# Autodesk Inventor assembly: SoporteBobina_1
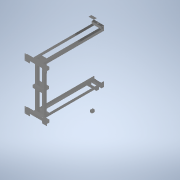
[picture p0: Inventor's stored thumbnail of the model, 180x180]
Saved by Autodesk Inventor 2022 (Build 260153000, 153)
## iProperties
Created: 2022-03-28
Part Number: SoporteBobina_1
Document SubType Name: Assembly
Designer: aarco
Author: aarco
## Documents named in this file (10)
- C:\Users\dovalle\OneDrive - ALTER TECHNOLOGY TÜV NORD, S.A.U\Escritorio\IDOM\REV_3\SoporteBobina_1.iam
- C:\Users\dovalle\OneDrive - ALTER TECHNOLOGY TÜV NORD, S.A.U\Escritorio\IDOM\REV_3\A_1012_40_4.ipt
- C:\Users\dovalle\OneDrive - ALTER TECHNOLOGY TÜV NORD, S.A.U\Escritorio\IDOM\REV_3\C_370_40_2.ipt
- C:\Users\dovalle\OneDrive - ALTER TECHNOLOGY TÜV NORD, S.A.U\Escritorio\IDOM\REV_3\C_156_40_2.ipt
- C:\Users\dovalle\OneDrive - ALTER TECHNOLOGY TÜV NORD, S.A.U\Escritorio\IDOM\REV_3\C_805_40_2.ipt
- C:\Users\dovalle\OneDrive - ALTER TECHNOLOGY TÜV NORD, S.A.U\Escritorio\IDOM\REV_3\Placa_Rueda_105x85_80x60_3.ipt
- C:\Users\dovalle\OneDrive - ALTER TECHNOLOGY TÜV NORD, S.A.U\Escritorio\IDOM\REV_3\C_156_40_20_2.ipt
- C:\Users\dovalle\OneDrive - ALTER TECHNOLOGY TÜV NORD, S.A.U\Escritorio\IDOM\REV_3\C_164_40_4.ipt
- C:\Users\dovalle\OneDrive - ALTER TECHNOLOGY TÜV NORD, S.A.U\Escritorio\IDOM\REV_3\C_45_35_2.ipt
- C:\Users\dovalle\OneDrive - ALTER TECHNOLOGY TÜV NORD, S.A.U\Escritorio\IDOM\REV_3\PlacaSTC-HH20.ipt
## Components (24 placed, 9 different names)
1. A_1012_40_4:1 — Rígido:25, Rígido:29, Coincidencia:6
2. C_370_40_2:1 — Rígido:16, Rígido:19, Rígido:20
3. A_1012_40_4:2 — Rígido:27, Coincidencia:2, Nivelación:2
4. C_370_40_2:2 — Rígido:17, Rígido:18, Rígido:21
5. C_156_40_2:1 — Rígido:1, Rígido:2
6. C_156_40_2:4 — Rígido:5
7. C_156_40_2:5 — Rígido:6
8. C_156_40_2:6 — Rígido:7
9. C_805_40_2:1 — Rígido:2, Rígido:6, Rígido:7
10. C_805_40_2:2 — Rígido:1, Rígido:5, Rígido:22, Rígido:23
11. A_1012_40_4:3 — Rígido:26, Rígido:28, Coincidencia:3, Nivelación:3
12. A_1012_40_4:4 — Rígido:24
13. Placa_Rueda_105x85_80x60_3:1 — Rígido:16
14. Placa_Rueda_105x85_80x60_3:2 — Rígido:17
15. Placa_Rueda_105x85_80x60_3:3 — Rígido:18
16. Placa_Rueda_105x85_80x60_3:4 — Rígido:19
17. C_156_40_20_2:1 — Rígido:20, Rígido:22, Rígido:24, Rígido:25
18. C_156_40_20_2:2 — Rígido:21, Rígido:23, Rígido:26, Rígido:27
19. C_164_40_4:1 — Rígido:29
20. C_164_40_4:2 — Rígido:28, Coincidencia:5
21. C_45_35_2:1 — Coincidencia:3, Nivelación:3, Nivelación:4
22. C_45_35_2:2 — Coincidencia:2, Nivelación:2, Nivelación:4, Rígido:30, Coincidencia:5
23. PlacaSTC-HH20:1 — Rígido:30
24. C_45_35_2:3 — Coincidencia:6
## Relationships (27: WeldJoint 20, Mate 4, Flush 3)
- Rígido:1 [WeldJoint]: C_156_40_2:1 ↔ C_805_40_2:2
- Rígido:2 [WeldJoint]: C_156_40_2:1 ↔ C_805_40_2:1
- Rígido:5 [WeldJoint]: C_156_40_2:4 ↔ C_805_40_2:2
- Rígido:6 [WeldJoint]: C_156_40_2:5 ↔ C_805_40_2:1
- Rígido:7 [WeldJoint]: C_156_40_2:6 ↔ C_805_40_2:1
- Rígido:16 [WeldJoint]: C_370_40_2:1 ↔ Placa_Rueda_105x85_80x60_3:1
- Rígido:17 [WeldJoint]: C_370_40_2:2 ↔ Placa_Rueda_105x85_80x60_3:2
- Rígido:18 [WeldJoint]: C_370_40_2:2 ↔ Placa_Rueda_105x85_80x60_3:3
- Rígido:19 [WeldJoint]: C_370_40_2:1 ↔ Placa_Rueda_105x85_80x60_3:4
- Rígido:20 [WeldJoint]: C_370_40_2:1 ↔ C_156_40_20_2:1
- Rígido:21 [WeldJoint]: C_370_40_2:2 ↔ C_156_40_20_2:2
- Rígido:22 [WeldJoint]: C_805_40_2:2 ↔ C_156_40_20_2:1
- Rígido:23 [WeldJoint]: C_805_40_2:2 ↔ C_156_40_20_2:2
- Rígido:24 [WeldJoint]: A_1012_40_4:4 ↔ C_156_40_20_2:1
- Rígido:25 [WeldJoint]: A_1012_40_4:1 ↔ C_156_40_20_2:1
- Rígido:26 [WeldJoint]: A_1012_40_4:3 ↔ C_156_40_20_2:2
- Rígido:27 [WeldJoint]: A_1012_40_4:2 ↔ C_156_40_20_2:2
- Rígido:28 [WeldJoint]: A_1012_40_4:3 ↔ C_164_40_4:2
- Rígido:29 [WeldJoint]: A_1012_40_4:1 ↔ C_164_40_4:1
- Coincidencia:2 [Mate]: A_1012_40_4:2 ↔ C_45_35_2:2
- Nivelación:2 [Flush]: A_1012_40_4:2 ↔ C_45_35_2:2
- Coincidencia:3 [Mate]: A_1012_40_4:3 ↔ C_45_35_2:1
- Nivelación:3 [Flush]: A_1012_40_4:3 ↔ C_45_35_2:1
- Nivelación:4 [Flush]: C_45_35_2:1 ↔ C_45_35_2:2
- Rígido:30 [WeldJoint]: C_45_35_2:2 ↔ PlacaSTC-HH20:1
- Coincidencia:5 [Mate] (39.5 mm): C_164_40_4:2 ↔ C_45_35_2:2
- Coincidencia:6 [Mate]: A_1012_40_4:1 ↔ C_45_35_2:3
